# Autodesk Inventor assembly: linkage_system_test_2
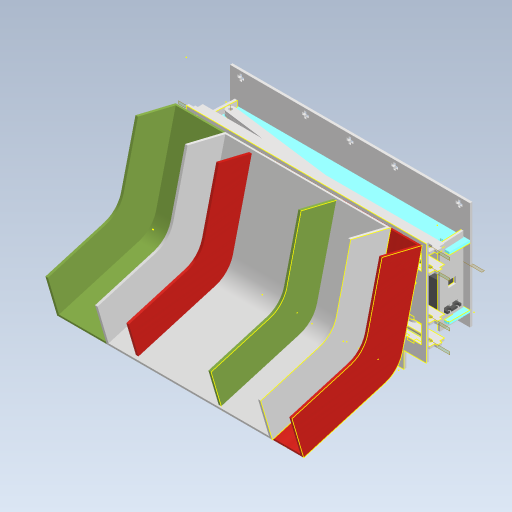
[picture p0: Inventor's stored thumbnail of the model, 512x512]
Saved by Autodesk Inventor 2023 (Build 270158000, 158)
## iProperties
Created: 2023-06-07
Part Number: linkage_system_test_2
Document SubType Name: Assembly
Designer: JOU
Author: JOU
## Documents named in this file (15)
- C:\Users\JOU\Desktop\git\Areo_Rider_Cabin\Expansion\test\linkage_system_test_2.iam
- C:\Users\JOU\Desktop\git\Areo_Rider_Cabin\Expansion\test\plate_expansion.ipt
- C:\Users\JOU\Desktop\git\Areo_Rider_Cabin\Expansion\test\零件1.ipt
- C:\Users\JOU\Desktop\git\Areo_Rider_Cabin\Expansion\test\零件8.ipt
- C:\Users\JOU\Desktop\git\Areo_Rider_Cabin\Expansion\test\零件4.ipt
- C:\Users\JOU\Desktop\git\Areo_Rider_Cabin\Expansion\test\零件5.ipt
- C:\Users\JOU\Desktop\git\Areo_Rider_Cabin\car\外抓檔\Tower Pro MG996R.ipt
- C:\Users\JOU\Desktop\git\Areo_Rider_Cabin\Expansion\test\adjustable_130.ipt
- C:\Users\JOU\Desktop\git\Areo_Rider_Cabin\Expansion\test\adjustable_200.ipt
- C:\Users\JOU\Desktop\git\Areo_Rider_Cabin\Expansion\test\零件12.ipt
- C:\Users\JOU\Desktop\git\Areo_Rider_Cabin\Expansion\test\adjustable_80.ipt
- C:\Users\JOU\Desktop\git\Areo_Rider_Cabin\Airfoil & Nuzzle\sus_1.ipt
- C:\Users\JOU\Desktop\git\Areo_Rider_Cabin\Airfoil & Nuzzle\sus_2.ipt
- C:\Users\JOU\Desktop\git\Areo_Rider_Cabin\Airfoil & Nuzzle\splitter.ipt
- C:\Users\JOU\Desktop\git\Areo_Rider_Cabin\Expansion\test\零件7.ipt
## Components (33 placed, 14 different names)
1. plate_expansion:1
2. 零件1:1
3. 零件8:1
4. 零件4:1 — 貼合:37, 貼合:38
5. 零件4:2 — 貼合:42
6. 零件4:3 — 貼合:39, 貼合:40
7. 零件4:4 — 貼合:41
8. 零件5:1 — 貼合:51, 貼合:52, 貼合:53, 貼合:54, 貼合:55, 貼合:56
9. 零件8:2
10. Tower Pro MG996R:1
11. Tower Pro MG996R:2
12. 零件1:2 — 貼合:36
13. adjustable_130:1 — 貼合:37, 貼合:38
14. adjustable_200:1 — 貼合:36
15. adjustable_200:2
16. adjustable_200:3 — 貼合:41
17. adjustable_200:4
18. adjustable_200:5 — 貼合:40
19. adjustable_200:6
20. adjustable_200:7 — 貼合:42
21. adjustable_200:8
22. 零件12:1
23. adjustable_80:1 — 貼合:39
24. adjustable_130:2
25. 零件12:2
26. adjustable_80:2
27. sus_1:1
28. sus_2:1 — 貼合:57
29. splitter:1
30. splitter:2
31. splitter:3
32. 零件7:1 — 貼合:51, 貼合:52, 貼合:53
33. 零件7:2 — 貼合:54, 貼合:55, 貼合:56, 貼合:57
## Relationships (76: Mate 45, Insert 19, Flush 11, Angle 1)
- [Mate]: plate_expansion:1 ↔ 零件1:1
- [Flush]: plate_expansion:1 ↔ 零件1:1
- [Mate]: plate_expansion:1 ↔ 零件1:1
- [Mate]: 零件1:1 ↔ 零件8:1
- [Mate]: 零件1:1 ↔ 零件8:1
- [Flush]: 零件4:2 ↔ 零件4:4
- [Flush]: 零件4:1 ↔ 零件4:2
- [Flush]: 零件4:1 ↔ 零件4:3
- [Flush]: 零件4:1 ↔ 零件5:1
- [Mate]: 零件4:1 ↔ 零件5:1
- [Mate]: 零件4:3 ↔ 零件5:1
- [Mate]: 零件4:2 ↔ 零件5:1
- [Mate]: 零件4:4 ↔ 零件5:1
- [Mate]: 零件4:3 ↔ 零件5:1
- [Angle] (0 deg): plate_expansion:1 ↔ 零件5:1
- [Flush]: plate_expansion:1 ↔ 零件5:1
- [Mate]: 零件1:1 ↔ 零件8:2
- [Insert]: 零件1:1 ↔ Tower Pro MG996R:2
- [Mate]: plate_expansion:1 ↔ 零件1:2
- [Flush]: plate_expansion:1 ↔ 零件1:2
- [Flush]: 零件1:1 ↔ 零件1:2
- [Insert]: Tower Pro MG996R:1 ↔ 零件1:2
- [Mate]: 零件8:1 ↔ Tower Pro MG996R:1
- [Mate]: 零件8:2 ↔ Tower Pro MG996R:2
- [Mate]: 零件1:1 ↔ 零件8:2
- [Mate]: 零件4:1 ↔ 零件5:1
- [Mate]: 零件4:2 ↔ 零件5:1
- [Mate]: 零件4:4 ↔ 零件5:1
- [Insert]: adjustable_200:1 ↔ adjustable_200:2
- [Insert]: adjustable_200:1 ↔ adjustable_200:2
- [Mate]: 零件1:2 ↔ adjustable_200:1
- [Insert]: adjustable_200:3 ↔ adjustable_200:4
- [Insert]: adjustable_200:3 ↔ adjustable_200:4
- [Insert]: adjustable_200:5 ↔ adjustable_200:6
- [Insert]: adjustable_200:5 ↔ adjustable_200:6
- [Insert]: adjustable_200:7 ↔ adjustable_200:8
- [Insert]: adjustable_200:7 ↔ adjustable_200:8
- [Mate]: Tower Pro MG996R:2 ↔ adjustable_200:4
- [Mate] (3.87 mm): 零件1:1 ↔ adjustable_200:3
- [Insert]: 零件1:1 ↔ adjustable_200:7
- [Mate]: Tower Pro MG996R:1 ↔ adjustable_200:6
- [Mate] (3.87 mm): 零件1:2 ↔ adjustable_200:6
- [Insert]: adjustable_80:1 ↔ 零件12:2
- [Insert]: adjustable_80:1 ↔ adjustable_130:2
- [Insert]: adjustable_200:6 ↔ 零件12:2
- [Insert]: adjustable_200:6 ↔ adjustable_130:2
- [Insert]: adjustable_200:1 ↔ 零件12:1
- [Insert]: adjustable_130:1 ↔ adjustable_200:1
- [Insert]: adjustable_130:1 ↔ adjustable_80:2
- [Insert]: 零件12:1 ↔ adjustable_80:2
- [Flush]: adjustable_130:1 ↔ adjustable_130:2
- [Mate]: 零件4:3 ↔ adjustable_200:5
- 貼合:36 [Mate] (3 mm): 零件1:2 ↔ adjustable_200:1
- 貼合:37 [Mate]: 零件4:1 ↔ adjustable_130:1
- 貼合:38 [Mate]: 零件4:1 ↔ adjustable_130:1
- 貼合:39 [Mate]: 零件4:3 ↔ adjustable_80:1
- 貼合:40 [Mate]: 零件4:3 ↔ adjustable_200:5
- 貼合:41 [Mate]: 零件4:4 ↔ adjustable_200:3
- 貼合:42 [Mate]: 零件4:2 ↔ adjustable_200:7
- [Mate]: splitter:2 ↔ splitter:3
- [Mate]: splitter:1 ↔ splitter:3
- [Mate]: splitter:2 ↔ splitter:3
- [Mate]: splitter:1 ↔ splitter:3
- [Mate]: sus_2:1 ↔ splitter:3
- [Mate]: sus_2:1 ↔ splitter:3
- [Mate]: sus_1:1 ↔ splitter:1
- [Mate]: sus_1:1 ↔ splitter:1
- [Flush] (20 mm): sus_2:1 ↔ splitter:3
- [Flush] (20 mm): sus_1:1 ↔ splitter:1
- 貼合:51 [Mate]: 零件5:1 ↔ 零件7:1
- 貼合:52 [Mate]: 零件5:1 ↔ 零件7:1
- 貼合:53 [Mate]: 零件5:1 ↔ 零件7:1
- 貼合:54 [Mate]: 零件5:1 ↔ 零件7:2
- 貼合:55 [Mate]: 零件5:1 ↔ 零件7:2
- 貼合:56 [Mate]: 零件5:1 ↔ 零件7:2
- 貼合:57 [Mate]: sus_2:1 ↔ 零件7:2
## Named parameters: d455_d451 = 0 mm, d456_d452 = 0 mm, d437_d433 = 0 mm, d438_d434 = 0 mm, d439_d437_d433 = 0 mm, d440_d438_d434 = 0 mm, d441_d437_d433 = 0 mm, d442_d438_d434 = 0 mm, d71_d66 = 0 mm, d72_d67 = 0 mm, d73_d68 = 0 mm, d74_d69 = 0 mm, d75_d70 = 0 mm
